# Autodesk Inventor assembly: fullSparFlat
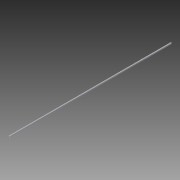
[picture p0: Inventor's stored thumbnail of the model, 180x180]
Saved by Autodesk Inventor 2014 (Build 180170000, 170)
## iProperties
Created: 2015-03-27
Part Number: fullSparFlat
Document SubType Name: Assembly
Designer: ddeboer
Author: ddeboer
## Documents named in this file (4)
- C:\Users\ddeboer\Desktop\hera-cad\surface\sparFullFlat.iam
- C:\Users\ddeboer\Desktop\hera-cad\surface\pvcSection_63mm.ipt
- C:\Users\ddeboer\Desktop\hera-cad\smallParts\coupler_63mm.ipt
- C:\Users\ddeboer\Desktop\hera-cad\surface\pvcSection_63mm_cut4full.ipt
## Components (3 placed, 3 different names)
1. pvcSection_63mm:2 — Insert:3
2. coupler_63mm:1 — Insert:3, Insert:4
3. pvcSection_63mm_cut4full:1 — Insert:4
## Relationships (2: Insert 2)
- Insert:3 (-29.3624 mm): pvcSection_63mm:2 ↔ coupler_63mm:1
- Insert:4 (-29.3624 mm): coupler_63mm:1 ↔ pvcSection_63mm_cut4full:1
